# Autodesk Inventor assembly: 足(単独)
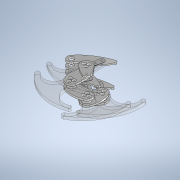
[picture p0: Inventor's stored thumbnail of the model, 180x180]
Saved by Autodesk Inventor 2022.2 (Build 262287000, 287)
## iProperties
Created: 2022-01-09
Part Number: 足(単独)
Document SubType Name: Assembly
Designer: acps
Author: acps
## Documents named in this file (3)
- C:\Users\acps\Documents\srdc\srdc_ksh\足(単独).iam
- C:\Users\acps\Documents\srdc\srdc_ksh\揺動節+ヘッケン.iam
- C:\Users\acps\Documents\srdc\srdc_ksh\クランク.iam
## Components (5 placed, 2 different names)
1. 揺動節+ヘッケン:1 [sub-assembly] — Mate:2, Insert:2, Mate:5, Mate:6, Mate:7
2. 揺動節+ヘッケン:2 [sub-assembly] — Mate:1, Insert:1, Mate:5
3. 揺動節+ヘッケン:3 [sub-assembly] — Mate:4, Insert:4, Mate:6
4. 揺動節+ヘッケン:4 [sub-assembly] — Mate:3, Insert:3, Mate:7
5. クランク:1 [sub-assembly] — Mate:1, Insert:1, Mate:2, Mate:3, Mate:4, Insert:2, Insert:3, Insert:4
## Relationships (11: Mate 7, Insert 4)
- Mate:1: 揺動節+ヘッケン:2 ↔ クランク:1
- Insert:1: 揺動節+ヘッケン:2 ↔ クランク:1
- Mate:2: 揺動節+ヘッケン:1 ↔ クランク:1
- Mate:3: 揺動節+ヘッケン:4 ↔ クランク:1
- Mate:4: 揺動節+ヘッケン:3 ↔ クランク:1
- Insert:2: 揺動節+ヘッケン:1 ↔ クランク:1
- Insert:3: 揺動節+ヘッケン:4 ↔ クランク:1
- Insert:4: 揺動節+ヘッケン:3 ↔ クランク:1
- Mate:5: 揺動節+ヘッケン:1 ↔ 揺動節+ヘッケン:2
- Mate:6: 揺動節+ヘッケン:1 ↔ 揺動節+ヘッケン:3
- Mate:7: 揺動節+ヘッケン:1 ↔ 揺動節+ヘッケン:4
